# Autodesk Inventor assembly: Tread Wheel Assembly
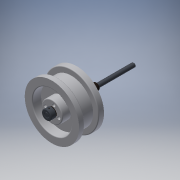
[picture p0: Inventor's stored thumbnail of the model, 180x180]
Saved by Autodesk Inventor 2016 (Build 200138000, 138)
## iProperties
Created: 2015-12-14
Part Number: Tread Wheel Assembly
Document SubType Name: Assembly
Designer: tbloo
Author: tbloo
## Documents named in this file (6)
- C:\Users\TimB\Documents\GitHub\phi_robotics\3d-models\FTC_Tetrix_KOP_Block_Party\Tim Bloot Designs\JAr JaR Bot\Tread Wheel Assembly.iam
- C:\Users\TimB\Documents\GitHub\phi_robotics\3d-models\FTC_Tetrix_KOP_Block_Party\Tetrix_Kit_FTC\Autodesk Inventor Files\tetrix_axle.ipt
- C:\Users\TimB\Documents\GitHub\phi_robotics\3d-models\FTC_Tetrix_KOP_Block_Party\Tetrix_Kit_FTC\Autodesk Inventor Files\tetrix_bushing.ipt
- C:\Users\TimB\Documents\GitHub\phi_robotics\3d-models\FTC_Tetrix_KOP_Block_Party\Tetrix_Kit_FTC\Autodesk Inventor Files\tetrix_tread_wheel.ipt
- C:\Users\TimB\Documents\GitHub\phi_robotics\3d-models\FTC_Tetrix_KOP_Block_Party\Tetrix_Kit_FTC\Autodesk Inventor Files\tetrix_739092_2012.iam
- C:\Users\TimB\Documents\GitHub\phi_robotics\3d-models\FTC_Tetrix_KOP_Block_Party\Tetrix_Kit_FTC\Autodesk Inventor Files\tetrix_axle_spacer-big.ipt
## Components (7 placed, 5 different names)
1. tetrix_axle:1 — Rigid:1, Rotational:4, Rotational:7
2. tetrix_bushing:3 — Rotational:6
3. tetrix_tread_wheel:1 — Rotational:5, Rotational:6
4. tetrix_bushing:4 — Rotational:4, Rotational:5
5. tetrix_739092_2012:1 [sub-assembly] — Rigid:1
6. tetrix_axle_spacer-big:1 — Rotational:7, Rotational:8
7. tetrix_bushing:5 — Rotational:8
## Relationships (6: RevoluteJoint 5, WeldJoint 1)
- Rigid:1 [WeldJoint]: tetrix_axle:1 ↔ tetrix_739092_2012:1
- Rotational:4 [RevoluteJoint] (-6.2 mm): tetrix_axle:1 ↔ tetrix_bushing:4
- Rotational:5 [RevoluteJoint]: tetrix_tread_wheel:1 ↔ tetrix_bushing:4
- Rotational:6 [RevoluteJoint]: tetrix_bushing:3 ↔ tetrix_tread_wheel:1
- Rotational:7 [RevoluteJoint] (-55.5 mm): tetrix_axle:1 ↔ tetrix_axle_spacer-big:1
- Rotational:8 [RevoluteJoint]: tetrix_axle_spacer-big:1 ↔ tetrix_bushing:5
